# Autodesk Inventor assembly: robot
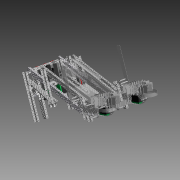
[picture p0: Inventor's stored thumbnail of the model, 180x180]
Saved by Autodesk Inventor 2014 SP1 (Build 180222100, 222)
## iProperties
Created: 2013-09-09
Part Number: robot
Document SubType Name: Assembly
Designer: Ryan
Author: Ryan
## Documents named in this file (9)
- C:\Users\Ryan\Desktop\sw\toss up 2ed A bot\manipulator\manipulator.iam
- C:\Users\Ryan\Desktop\sw\toss up 2ed A bot\toss up tower\encoder metal assembly.iam
- C:\Users\Ryan\Desktop\sw\toss up 2ed A bot\toss up tower\triangle support.iam
- C:\Users\Ryan\Desktop\sw\toss up 2ed A bot\toss up tower\triangle support_MIR.iam
- C:\Users\Ryan\Desktop\sw\toss up 2ed A bot\6 bar\6 bar.iam
- C:\Users\Ryan\Desktop\sw\toss up 2ed A bot\6 bar\6 bar_MIR.iam
- C:\Users\Ryan\Desktop\sw\toss up 2ed A bot\toss up tower\cortex plate.iam
- C:\Users\Ryan\Desktop\sw\toss up 2ed A bot\toss up tower\tower1.iam
- C:\Users\Ryan\Desktop\sw\toss up 2ed A bot\intake\full intake.iam
## Components (9 placed, 8 different names)
1. 6 bar:1 [sub-assembly] — Mate:13, Flush:52, Mate:14, Mate:15, Mate:16, Mate:25, Angle:2
2. 6 bar_MIR:1 [sub-assembly] — Mate:8, Mate:9, Mate:10, Mate:11, Flush:52, Mate:20, Mate:21, Mate:22, Mate:24, Angle:2
3. cortex plate:1 [sub-assembly] — Mate:27, Flush:54, Flush:55
4. tower1:1 [sub-assembly] — Mate:13, Mate:14, Mate:15, Mate:16, Mate:23, Mate:25
5. tower1:2 [sub-assembly] — Mate:3, Mate:4, Mate:5, Mate:6, Mate:8, Mate:9, Mate:10, Mate:11, Mate:17, Mate:18, Angle:1, Mate:24, Flush:53, Mate:26, Mate:27, Flush:54, Flush:55
6. full intake:1 [sub-assembly] — Mate:20, Mate:21, Mate:22
7. encoder metal assembly:1 [sub-assembly] — Mate:3, Mate:4, Mate:5, Mate:6
8. triangle support:1 [sub-assembly] — Flush:40, Flush:41, Mate:17, Mate:18, Angle:1, Flush:53, Mate:26
9. triangle support_MIR:1 [sub-assembly] — Flush:40, Flush:41, Mate:23
## Relationships (30: Mate 22, Flush 6, Angle 2)
- Flush:40: triangle support:1 ↔ triangle support_MIR:1
- Flush:41: triangle support:1 ↔ triangle support_MIR:1
- Mate:3: tower1:2 ↔ encoder metal assembly:1
- Mate:4 (2.3114 mm): tower1:2 ↔ encoder metal assembly:1
- Mate:5 (2.3114 mm): tower1:2 ↔ encoder metal assembly:1
- Mate:6 (2.3114 mm): tower1:2 ↔ encoder metal assembly:1
- Mate:8: 6 bar_MIR:1 ↔ tower1:2
- Mate:9 (2.3114 mm): 6 bar_MIR:1 ↔ tower1:2
- Mate:10 (2.3114 mm): 6 bar_MIR:1 ↔ tower1:2
- Mate:11 (2.3114 mm): 6 bar_MIR:1 ↔ tower1:2
- Mate:13: 6 bar:1 ↔ tower1:1
- Flush:52: 6 bar:1 ↔ 6 bar_MIR:1
- Mate:14 (2.3114 mm): 6 bar:1 ↔ tower1:1
- Mate:15 (2.3114 mm): 6 bar:1 ↔ tower1:1
- Mate:16 (2.3114 mm): 6 bar:1 ↔ tower1:1
- Mate:17: tower1:2 ↔ triangle support:1
- Mate:18 (2.3114 mm): tower1:2 ↔ triangle support:1
- Angle:1 (0 deg): tower1:2 ↔ triangle support:1
- Mate:20: 6 bar_MIR:1 ↔ full intake:1
- Mate:21: 6 bar_MIR:1 ↔ full intake:1
- Mate:22: 6 bar_MIR:1 ↔ full intake:1
- Mate:23: tower1:1 ↔ triangle support_MIR:1
- Mate:24: 6 bar_MIR:1 ↔ tower1:2
- Mate:25: 6 bar:1 ↔ tower1:1
- Angle:2 (0 deg): 6 bar:1 ↔ 6 bar_MIR:1
- Flush:53 (-20.0914 mm): tower1:2 ↔ triangle support:1
- Mate:26 (2.3114 mm): tower1:2 ↔ triangle support:1
- Mate:27 (3.175 mm): cortex plate:1 ↔ tower1:2
- Flush:54: cortex plate:1 ↔ tower1:2
- Flush:55: cortex plate:1 ↔ tower1:2
## Named parameters: q = 2.3114 mm
